# Autodesk Inventor assembly: SyringeConcept1
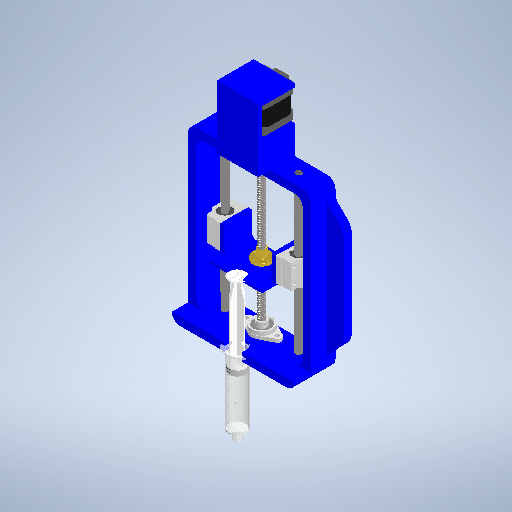
[picture p0: Inventor's stored thumbnail of the model, 512x512]
Saved by Autodesk Inventor 2025.2 (Build 292293000, 293)
## iProperties
Created: 2025-05-30
Part Number: SyringeConcept1
Document SubType Name: Assembly
Designer: Simon
Author: Simon
## Documents named in this file (13)
- C:\Users\Simon\OneDrive\Documents\Inventor\Skripsie2025\Extruder Concept 2\SyringeConcept2.iam
- C:\Users\Simon\OneDrive\Documents\Inventor\Skripsie2025\PartsFolder\Syringe\Rubber tampon_20ml.ipt
- C:\Users\Simon\OneDrive\Documents\Inventor\Skripsie2025\PartsFolder\Syringe\Syringe_cylinder_20ml.ipt
- C:\Users\Simon\OneDrive\Documents\Inventor\Skripsie2025\PartsFolder\Syringe\Syringe_piston_20ml.ipt
- C:\Users\Simon\OneDrive\Documents\Inventor\Skripsie2025\Extruder Concept 2\Frame.ipt
- C:\Users\Simon\OneDrive\Documents\Inventor\Skripsie2025\Extruder Concept 2\TR8x8-4_LeadScrew_200mm.ipt
- C:\Users\Simon\OneDrive\Documents\Inventor\Skripsie2025\PartsFolder\Flexible Coupling 5,8.ipt
- C:\Users\Simon\OneDrive\Documents\Inventor\Skripsie2025\PartsFolder\Pillow Block Bearing 1\Zinc Alloy Pillow Block Flange Bearing KFL08 ID-8mm.iam
- C:\Users\Simon\OneDrive\Documents\Inventor\Skripsie2025\PartsFolder\Stepper_17HS4401.ipt
- C:\Users\Simon\OneDrive\Documents\Inventor\Skripsie2025\PartsFolder\TR8x8-4_Nut.ipt
- C:\Users\Simon\OneDrive\Documents\Inventor\Skripsie2025\PartsFolder\SC8UU\SC8UU.iam
- C:\Users\Simon\OneDrive\Documents\Inventor\Skripsie2025\Extruder Concept 2\SteelShaft_195mm.ipt
- C:\Users\Simon\OneDrive\Documents\Inventor\Skripsie2025\Extruder Concept 2\SyringePushMount.ipt
## Components (14 placed, 12 different names)
1. Rubber tampon_20ml:1 — Mate:1, Mate:2
2. Syringe_cylinder_20ml:1 — Mate:3, Mate:26, Angle:5, Mate:27
3. Syringe_piston_20ml:1 — Mate:1, Mate:2, Mate:3, Angle:6, Mate:34
4. Frame:1 — Mate:4, Mate:5, Mate:6, Mate:7, Mate:8, Mate:9, Mate:10, Mate:13, Mate:20, Mate:21, Angle:2, Angle:3, Angle:4, Mate:26, Angle:5, Mate:27, Angle:6
5. TR8x8-4_LeadScrew_200mm:1 — Mate:14, Flush:2, Mate:15, Mate:16, Mate:17, Mate:19, Mate:28
6. Flexible Coupling 5,8:1 — Mate:16, Mate:17, Mate:18
7. Zinc Alloy Pillow Block Flange Bearing KFL08 ID-8mm:1 [sub-assembly] — Mate:13, Mate:14, Flush:2, Mate:20, Mate:21
8. Stepper_17HS4401:1 — Mate:18, Mate:19, Angle:4
9. TR8x8-4_Nut:1 — Mate:15, Mate:32, Mate:33
10. SC8UU:1 [sub-assembly] — Mate:12, Angle:1, Flush:1, Mate:31
11. SC8UU:2 [sub-assembly] — Mate:11, Angle:1, Flush:1, Angle:2, Mate:29, Mate:30
12. SteelShaft_195mm:1 — Mate:7, Mate:10, Mate:12
13. SteelShaft_195mm:2 — Mate:8, Mate:9, Mate:11
14. SyringePushMount:1 — Angle:3, Mate:28, Mate:29, Mate:30, Mate:31, Mate:32, Mate:33, Mate:34
## Relationships (38: Mate 30, Angle 6, Flush 2)
- Mate:1: Rubber tampon_20ml:1 ↔ Syringe_piston_20ml:1
- Mate:2: Rubber tampon_20ml:1 ↔ Syringe_piston_20ml:1
- Mate:3: Syringe_cylinder_20ml:1 ↔ Syringe_piston_20ml:1
- Mate:4: Frame:1
- Mate:5: Frame:1
- Mate:6: Frame:1
- Mate:7: Frame:1 ↔ SteelShaft_195mm:1
- Mate:8: Frame:1 ↔ SteelShaft_195mm:2
- Mate:9: Frame:1 ↔ SteelShaft_195mm:2
- Mate:10: Frame:1 ↔ SteelShaft_195mm:1
- Mate:11: SC8UU:2 ↔ SteelShaft_195mm:2
- Mate:12: SC8UU:1 ↔ SteelShaft_195mm:1
- Angle:1 (180 deg): SC8UU:1 ↔ SC8UU:2
- Flush:1: SC8UU:1 ↔ SC8UU:2
- Mate:13: Frame:1 ↔ Zinc Alloy Pillow Block Flange Bearing KFL08 ID-8mm:1
- Mate:14: TR8x8-4_LeadScrew_200mm:1 ↔ Zinc Alloy Pillow Block Flange Bearing KFL08 ID-8mm:1
- Flush:2 (2 mm): TR8x8-4_LeadScrew_200mm:1 ↔ Zinc Alloy Pillow Block Flange Bearing KFL08 ID-8mm:1
- Mate:15: TR8x8-4_LeadScrew_200mm:1 ↔ TR8x8-4_Nut:1
- Mate:16: TR8x8-4_LeadScrew_200mm:1 ↔ Flexible Coupling 5,8:1
- Mate:17: TR8x8-4_LeadScrew_200mm:1 ↔ Flexible Coupling 5,8:1
- Mate:18: Flexible Coupling 5,8:1 ↔ Stepper_17HS4401:1
- Mate:19: TR8x8-4_LeadScrew_200mm:1 ↔ Stepper_17HS4401:1
- Mate:20: Frame:1 ↔ Zinc Alloy Pillow Block Flange Bearing KFL08 ID-8mm:1
- Mate:21: Frame:1 ↔ Zinc Alloy Pillow Block Flange Bearing KFL08 ID-8mm:1
- Angle:2 (0 deg): Frame:1 ↔ SC8UU:2
- Angle:3 (0 deg): Frame:1 ↔ SyringePushMount:1
- Angle:4 (0 deg): Frame:1 ↔ Stepper_17HS4401:1
- Mate:26: Syringe_cylinder_20ml:1 ↔ Frame:1
- Angle:5 (0 deg): Syringe_cylinder_20ml:1 ↔ Frame:1
- Mate:27: Syringe_cylinder_20ml:1 ↔ Frame:1
- Mate:28: TR8x8-4_LeadScrew_200mm:1 ↔ SyringePushMount:1
- Mate:29: SC8UU:2 ↔ SyringePushMount:1
- Mate:30: SC8UU:2 ↔ SyringePushMount:1
- Mate:31: SC8UU:1 ↔ SyringePushMount:1
- Mate:32: TR8x8-4_Nut:1 ↔ SyringePushMount:1
- Mate:33: TR8x8-4_Nut:1 ↔ SyringePushMount:1
- Angle:6 (0 deg): Syringe_piston_20ml:1 ↔ Frame:1
- Mate:34: Syringe_piston_20ml:1 ↔ SyringePushMount:1
